# Autodesk Inventor assembly: AssyCage
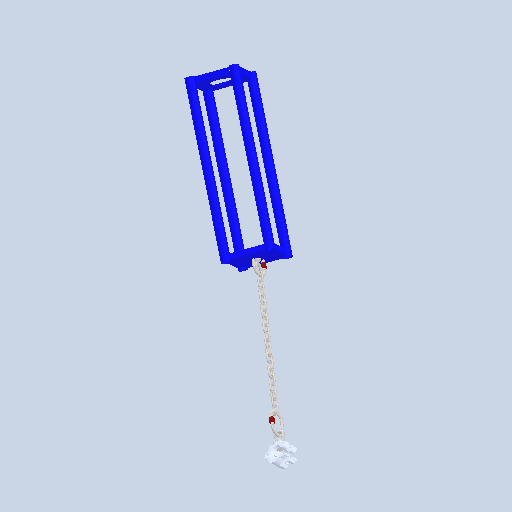
[picture p0: Inventor's stored thumbnail of the model, 512x512]
Saved by Autodesk Inventor 2025.2 (Build 292293000, 293)
## iProperties
Created: 2025-03-19
Part Number: AssyCage
Document SubType Name: Assembly
Designer: jings
Author: jings
## Documents named in this file (3)
- C:\Users\Baz Robotics\Downloads\2025-Poseidon-Mechanical\AssyCage.iam
- C:\Users\Baz Robotics\Downloads\2025-Poseidon-Mechanical\CageNoChain.ipt
- C:\Users\Baz Robotics\Downloads\2025-Poseidon-Mechanical\CageChainOnly.ipt
## Components (2 placed, 2 different names)
1. CageNoChain:1 — Tangent:1
2. CageChainOnly:1 — Tangent:1
## Relationships (1: Tangent 1)
- Tangent:1: CageNoChain:1 ↔ CageChainOnly:1
